# Autodesk Inventor assembly: assy
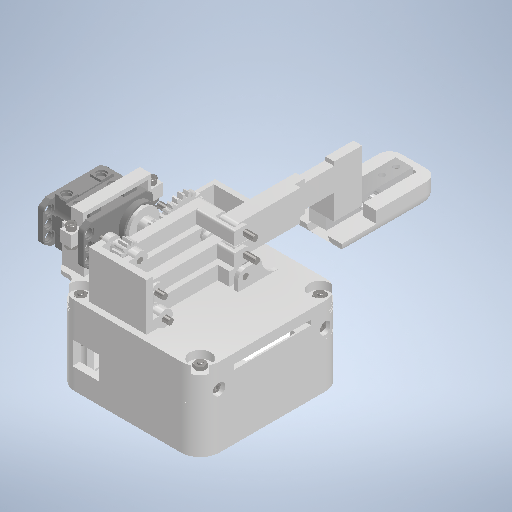
[picture p0: Inventor's stored thumbnail of the model, 512x512]
Saved by Autodesk Inventor 2025 (Build 290162000, 162)
## iProperties
Created: 2025-10-20
Part Number: assy
Document SubType Name: Assembly
Designer: sooo1
Author: sooo1
## Documents named in this file (4)
- C:\Users\sooo1\Downloads\final-20260216T060151Z-1-001\final\MOBITOUCH.iam
- C:\Users\sooo1\Downloads\final-20260216T060151Z-1-001\final\mobile_robot\mobile_robot.iam
- C:\Users\sooo1\Downloads\final-20260216T060151Z-1-001\final\stroke_module\adapter_tof.ipt
- C:\Users\sooo1\Downloads\final-20260216T060151Z-1-001\final\stroke_module\stroke_module.iam
## Components (4 placed, 3 different names)
1. adapter_tof:1
2. mobile_robot:1 [sub-assembly] — フラッシュ:1, フラッシュ:2, フラッシュ:3, メイト:1, メイト:2, メイト:3, メイト:4, メイト:5, メイト:6
3. stroke_module:1 [sub-assembly] — メイト:1, メイト:2, メイト:3
4. stroke_module:2 [sub-assembly] — メイト:4, メイト:5, メイト:6
## Relationships (9: Mate 6, Flush 3)
- フラッシュ:1 [Flush]: mobile_robot:1
- フラッシュ:2 [Flush]: mobile_robot:1
- フラッシュ:3 [Flush]: mobile_robot:1
- メイト:1 [Mate]: mobile_robot:1 ↔ stroke_module:1
- メイト:2 [Mate]: mobile_robot:1 ↔ stroke_module:1
- メイト:3 [Mate]: mobile_robot:1 ↔ stroke_module:1
- メイト:4 [Mate]: mobile_robot:1 ↔ stroke_module:2
- メイト:5 [Mate]: mobile_robot:1 ↔ stroke_module:2
- メイト:6 [Mate]: mobile_robot:1 ↔ stroke_module:2
